# Autodesk Inventor assembly: Tower
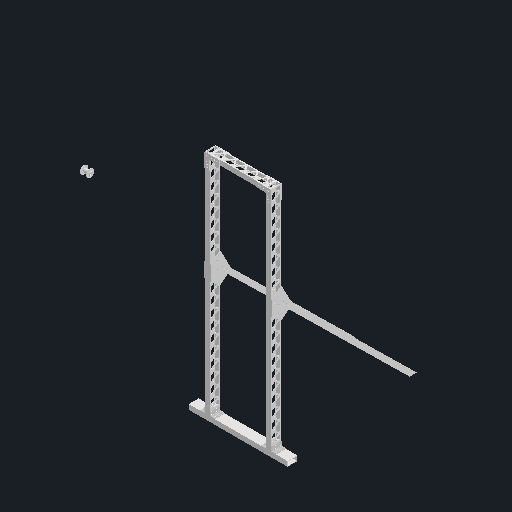
[picture p0: Inventor's stored thumbnail of the model, 512x512]
Saved by Autodesk Inventor 2023 (Build 270158000, 158)
## iProperties
Created: 2023-01-19
Part Number: Tower
Document SubType Name: Assembly
Designer: Terrence
Mass: 2797.17 g
Surface Area: 7389.26 cm^2
Volume: 1043.68 cm^3
Density: 2.6801 g/cm^3
Author: Terrence
## Documents named in this file (9)
- C:\Users\Terrence\Documents\FRC Long\Tower\Tower.iam
- C:\Users\Terrence\Documents\FRC Long\Tower\Solid1.ipt
- C:\Users\Terrence\Documents\FRC Long\Tower\Solid2.ipt
- C:\Users\Terrence\Documents\FRC Long\Tower\Solid3.ipt
- C:\Users\Terrence\Documents\FRC Long\Tower\Solid4.ipt
- C:\Users\Terrence\Documents\FRC Long\Tower\Solid6.ipt
- C:\Users\Terrence\Documents\FRC Long\Tower\am-4647_2000 Full Winch Spool For 2 in. Box Tube.ipt
- C:\Users\Terrence\Documents\FRC Long\Tower\Solid8.ipt
- C:\Users\Terrence\Documents\FRC Long\Tower\Solid7.ipt
## Components (19 placed, 8 different names)
1. Solid1:1 — Insert:1, Insert:2, Insert:3, Insert:4, Insert:13, Insert:14, Insert:17, Insert:18
2. Solid2:1 — Insert:5, Insert:6, Insert:11, Insert:12
3. Solid3:1 — Insert:15, Insert:16, Insert:22
4. Solid4:1 — Insert:3, Insert:4, Insert:5, Insert:6
5. Solid4:2 — Insert:1, Insert:2
6. Solid4:4 — Insert:7, Insert:8, Insert:11, Insert:12
7. Solid1:2 — Insert:7, Insert:8, Insert:9, Insert:10, Insert:19, Insert:20, Insert:21, Insert:33, Insert:34
8. Solid4:5 — Insert:9, Insert:10
9. Solid6:1 — Insert:13, Insert:14, Insert:15, Insert:16
10. Solid6:2 — Insert:17, Insert:18
11. Solid6:3 — Insert:19, Insert:20
12. Solid6:4 — Insert:21, Insert:22
13. am-4647_2000 Full Winch Spool For 2 in. Box Tube:1
14. Solid8:1 — Insert:25, Insert:26
15. Solid7:1 — Insert:25, Insert:26
16. Solid8:2
17. Solid8:3
18. Solid7:2 — Insert:31, Insert:32
19. Solid8:4 — Insert:31, Insert:32, Insert:33, Insert:34
## Relationships (30: Insert 30)
- Insert:1: Solid1:1 ↔ Solid4:2
- Insert:2: Solid1:1 ↔ Solid4:2
- Insert:3: Solid1:1 ↔ Solid4:1
- Insert:4: Solid1:1 ↔ Solid4:1
- Insert:5: Solid2:1 ↔ Solid4:1
- Insert:6: Solid2:1 ↔ Solid4:1
- Insert:7: Solid4:4 ↔ Solid1:2
- Insert:8: Solid4:4 ↔ Solid1:2
- Insert:9: Solid1:2 ↔ Solid4:5
- Insert:10: Solid1:2 ↔ Solid4:5
- Insert:11: Solid2:1 ↔ Solid4:4
- Insert:12: Solid2:1 ↔ Solid4:4
- Insert:13: Solid1:1 ↔ Solid6:1
- Insert:14: Solid1:1 ↔ Solid6:1
- Insert:15: Solid3:1 ↔ Solid6:1
- Insert:16: Solid3:1 ↔ Solid6:1
- Insert:17: Solid1:1 ↔ Solid6:2
- Insert:18: Solid1:1 ↔ Solid6:2
- Insert:19: Solid1:2 ↔ Solid6:3
- Insert:20: Solid1:2 ↔ Solid6:3
- Insert:21: Solid1:2 ↔ Solid6:4
- Insert:22: Solid3:1 ↔ Solid6:4
- Insert:25: Solid8:1 ↔ Solid7:1
- Insert:26: Solid8:1 ↔ Solid7:1
- [Insert]: Solid8:3 ↔ Solid7:2
- [Insert]: Solid8:3 ↔ Solid7:2
- Insert:31: Solid7:2 ↔ Solid8:4
- Insert:32: Solid7:2 ↔ Solid8:4
- Insert:33: Solid1:2 ↔ Solid8:4
- Insert:34: Solid1:2 ↔ Solid8:4
## Named parameters: d28_d24 = 0 mm, d29_d25 = 0 mm
